# Autodesk Inventor assembly: PerfboardSandwichPrinthead
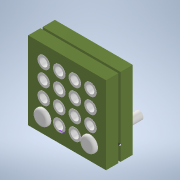
[picture p0: Inventor's stored thumbnail of the model, 180x180]
Saved by Autodesk Inventor 2021 (Build 250183000, 183)
## iProperties
Created: 2022-02-02
Part Number: PerfboardSandwichPrinthead
Document SubType Name: Assembly
Designer: Unit-005
Author: Unit-005
## Documents named in this file (5)
- C:\Users\Unit-005\Documents\Inventor\SiC_Monofilament_MicroheaterPrinthead\PerfboardSandwichPrinthead.iam
- C:\Users\Unit-005\Documents\Inventor\SiC_Monofilament_MicroheaterPrinthead\1.27mmpitchProtoboardDesign.ipt_.25inch_.25Inch.ipt
- C:\Users\Unit-005\Documents\Inventor\SiC_Monofilament_MicroheaterPrinthead\m0.6screw_4mm.ipt
- C:\Users\Unit-005\Documents\Inventor\SiC_Monofilament_MicroheaterPrinthead\4mmSicFilamentePerfBoard.ipt
- C:\Users\Unit-005\Documents\Inventor\SiC_Monofilament_MicroheaterPrinthead\1.27mmpitchProtoboardDesign.ipt_.25inch_.25Inch_MIR1.ipt
## Components (5 placed, 4 different names)
1. 4mmSicFilamentePerfBoard:1 — Tangent:1, Flush:1, Mate:1
2. 1.27mmpitchProtoboardDesign.ipt_.25inch_.25Inch:2 — Tangent:1, Flush:1, Mate:1, Mate:3, Mate:5, Mate:6, Mate:7
3. m0.6screw_4mm:1 — Mate:3, Mate:6
4. 1.27mmpitchProtoboardDesign.ipt_.25inch_.25Inch_MIR1:1
5. m0.6screw_4mm:2 — Mate:5, Mate:7
## Relationships (7: Mate 5, Tangent 1, Flush 1)
- Tangent:1 (0.006 mm): 4mmSicFilamentePerfBoard:1 ↔ 1.27mmpitchProtoboardDesign.ipt_.25inch_.25Inch:2
- Flush:1: 4mmSicFilamentePerfBoard:1 ↔ 1.27mmpitchProtoboardDesign.ipt_.25inch_.25Inch:2
- Mate:1: 4mmSicFilamentePerfBoard:1 ↔ 1.27mmpitchProtoboardDesign.ipt_.25inch_.25Inch:2
- Mate:3: 1.27mmpitchProtoboardDesign.ipt_.25inch_.25Inch:2 ↔ m0.6screw_4mm:1
- Mate:5: 1.27mmpitchProtoboardDesign.ipt_.25inch_.25Inch:2 ↔ m0.6screw_4mm:2
- Mate:6: 1.27mmpitchProtoboardDesign.ipt_.25inch_.25Inch:2 ↔ m0.6screw_4mm:1
- Mate:7: 1.27mmpitchProtoboardDesign.ipt_.25inch_.25Inch:2 ↔ m0.6screw_4mm:2
